# Autodesk Inventor assembly: Molde_levelled
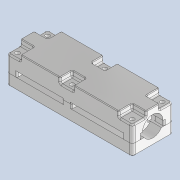
[picture p0: Inventor's stored thumbnail of the model, 180x180]
Saved by Autodesk Inventor 2020.4 (Build 244396000, 396)
## iProperties
Created: 2021-05-07
Part Number: Molde_levelled
Document SubType Name: Assembly
Designer: Acer
Author: Acer
## Documents named in this file (3)
- G:\Meu Drive\RobôCIn\Mecânica\SSL\2021\vRoboCup2021\first_floor\dribbler-3-gears\Molde_levelled.iam
- G:\Meu Drive\RobôCIn\Mecânica\SSL\2021\vRoboCup2021\first_floor\dribbler-3-gears\MoldeB_leveled.ipt
- G:\Meu Drive\RobôCIn\Mecânica\SSL\2021\vRoboCup2021\first_floor\dribbler-3-gears\MoldeA_leveled.ipt
## Components (2 placed, 1 different names)
1. Dribblerschnecke:1 — Mate:1, Mate:2, Mate:3
2. Dribblerschnecke:2 — Mate:1, Mate:2, Mate:3
## Relationships (3: Mate 3)
- Mate:1: Dribblerschnecke:1 ↔ Dribblerschnecke:2
- Mate:2: Dribblerschnecke:1 ↔ Dribblerschnecke:2
- Mate:3: Dribblerschnecke:1 ↔ Dribblerschnecke:2
